# Autodesk Inventor assembly: FA[23]
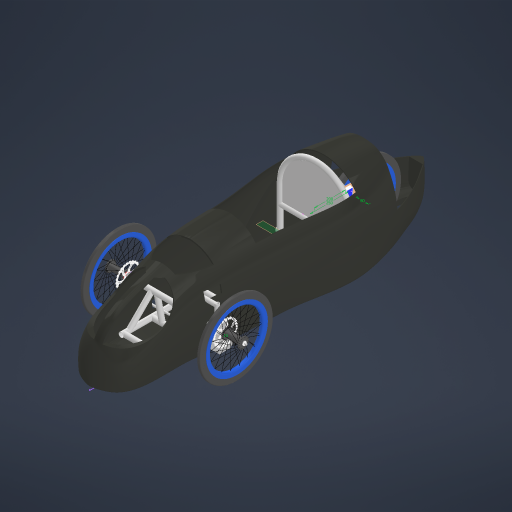
[picture p0: Inventor's stored thumbnail of the model, 512x512]
Saved by Autodesk Inventor 2024 (Build 280153000, 153)
## iProperties
Created: 2023-01-27
Part Number: FA[23]
Document SubType Name: Assembly
Designer: juanj
Author: juanj
## Documents named in this file (22)
- C:\Users\juanj\Documents\Documentos\Unisabana\Shell\A23[F]\FA[23].iam
- C:\Users\juanj\Documents\Documentos\Unisabana\Shell\A23[F]\PFA23[F]\FB23[F].ipt
- C:\Users\juanj\Documents\Documentos\Unisabana\Shell\A23[F]\PFA23[F]\TW23[F].ipt
- C:\Users\juanj\Documents\Documentos\Unisabana\Shell\A23[F]\PFA23[F]\W23[F].ipt
- C:\Users\juanj\Documents\Documentos\Unisabana\Shell\A23[F]\PFA23[F]\BU23[F].ipt
- C:\Users\juanj\Documents\Documentos\Unisabana\Shell\A23[F]\PFA23[F]\C23[F].ipt
- C:\Users\juanj\Documents\Documentos\Unisabana\Shell\A23[F]\PFA23[F]\R23[F].ipt
- C:\Users\juanj\Documents\Documentos\Unisabana\Shell\A23[F]\PFA23[F]\S23[F].ipt
- C:\Users\juanj\Documents\Documentos\Unisabana\Shell\A23[F]\PFA23[F]\N23[1][F].ipt
- C:\Users\juanj\Documents\Documentos\Unisabana\Shell\A23[F]\PFA23[F]\N23[F][2].ipt
- C:\Users\juanj\Documents\Documentos\Unisabana\Shell\A23[F]\PFA23[F]\D23[F].iam
- C:\Users\juanj\Documents\Documentos\Unisabana\Shell\A23[F]\PFA23[F]\M23[F].ipt
- C:\Users\juanj\Documents\Documentos\Unisabana\Shell\A23[F]\PFA23[F]\ET23[F].iam
- C:\Users\juanj\Documents\Documentos\Unisabana\Shell\A23[F]\PFA23[F]\BW23[F].ipt
- C:\Users\juanj\Documents\Documentos\Unisabana\Shell\C23 DESING\A23[F]\PFA23[F]\B23[F]_MIR2.ipt
- C:\Users\juanj\Documents\Documentos\Unisabana\Shell\C23 DESING\A23[F]\PFA23[F]\B23[F1].ipt
- C:\Users\juanj\Documents\Documentos\Unisabana\Shell\C23 DESING\A23[F]\PFA23[F]\HB[F].ipt
- C:\Users\juanj\Documents\Documentos\Unisabana\Shell\C23 DESING\A23[F]\PFA23[F]\C23[i3][L][2].ipt
- C:\Users\juanj\Documents\Documentos\Unisabana\Shell\C23 DESING\A23[F]\PFA23[F]\C23[i3][R][1].ipt
- C:\Users\juanj\Documents\Documentos\Unisabana\Shell\C23 DESING\A23[F]\PFA23[F]\DC23[L][F][1].ipt
- C:\Users\juanj\Documents\Documentos\Unisabana\Shell\C23 DESING\A23[F]\PFA23[F]\DC23[R][F][1].ipt
- C:\Users\juanj\Documents\Documentos\Unisabana\Shell\C23 DESING\A23[F]\PFA23[F]\SW23[F].ipt
## Components (30 placed, 21 different names)
1. C23[F]:1 — Insertar:3
2. FB23[F]:1 — Insertar:3, Insertar:4, Insertar:5, Insertar:6, Insertar:7, Insertar:8, Insertar:37, Nivelación:3, Nivelación:4, Insertar:38, Ángulo:8, Nivelación:5
3. TW23[F]:1 — Insertar:4
4. W23[F]:1 — Insertar:14
5. BU23[F]:1 — Insertar:14, Insertar:21, Insert:47
6. BU23[F]:2 — Insertar:15, Insertar:20, Insert:54
7. R23[F]:1 — Insertar:5, Insert:53
8. R23[F]:2 — Insertar:6
9. R23[F]:3 — Insertar:7
10. R23[F]:4 — Insertar:8, Insert:61
11. W23[F]:2 — Insertar:15
12. S23[F]:1 — Insert:43
13. S23[F]:2 — Insert:49
14. BW23[F]:1 — Insertar:38, Ángulo:8
15. ET23[F]:1 [sub-assembly] — Coincidencia:2, Coincidencia:3, Nivelación:6
16. M23[F]:1 — Insertar:37
17. D23[F]:1 [sub-assembly] — Insert:59, Mate:5
18. N23[F][2]:2 — Insertar:20
19. N23[1][F]:2 — Insert:51
20. N23[F][2]:1 — Insertar:21
21. N23[1][F]:1 — Insert:44
22. HB[F]:1 — Insert:58, Angle:18
23. C23[i3][L][2]:1 — Angle:11, Insert:41, Insert:43, Insert:47, Insert:53, Insert:60, Angle:20
24. C23[i3][R][1]:1 — Insert:49, Angle:14, Insert:50, Insert:54, Angle:17, Insert:61
25. DC23[L][F][1]:1 — Angle:11, Insert:41, Insert:44, Insert:55, Angle:16, Insert:59
26. DC23[R][F][1]:1 — Angle:14, Insert:50, Insert:51, Insert:56, Mate:5
27. B23[F]_MIR2:1 — Insert:56, Angle:17, Insert:58, Angle:18
28. B23[F1]:2 — Insert:55, Angle:16, Insert:57, Angle:19
29. HB[F]:3 — Insert:57, Angle:19
30. SW23[F]:1 — Insert:60, Angle:20
## Relationships (43: Insert 28, Angle 8, Flush 4, Mate 3)
- Insertar:3: C23[F]:1 ↔ FB23[F]:1
- Insertar:4: FB23[F]:1 ↔ TW23[F]:1
- Insertar:5: FB23[F]:1 ↔ R23[F]:1
- Insertar:6: FB23[F]:1 ↔ R23[F]:2
- Insertar:7: FB23[F]:1 ↔ R23[F]:3
- Insertar:8: FB23[F]:1 ↔ R23[F]:4
- Insertar:14: W23[F]:1 ↔ BU23[F]:1
- Insertar:15: BU23[F]:2 ↔ W23[F]:2
- Insertar:20: BU23[F]:2 ↔ N23[F][2]:2
- Insertar:21: BU23[F]:1 ↔ N23[F][2]:1
- Insertar:37: FB23[F]:1 ↔ M23[F]:1
- Nivelación:3 [Flush] (30 mm): FB23[F]:1
- Nivelación:4 [Flush] (29 mm): FB23[F]:1
- Coincidencia:2 [Mate]: ET23[F]:1
- Coincidencia:3 [Mate]: ET23[F]:1
- Insertar:38 (106.5 mm): FB23[F]:1 ↔ BW23[F]:1
- Ángulo:8 [Angle] (180 deg): FB23[F]:1 ↔ BW23[F]:1
- Nivelación:5 [Flush] (-50 mm): FB23[F]:1
- Nivelación:6 [Flush]: ET23[F]:1
- Angle:11 (0 deg): C23[i3][L][2]:1 ↔ DC23[L][F][1]:1
- Insert:41: C23[i3][L][2]:1 ↔ DC23[L][F][1]:1
- Insert:43: S23[F]:1 ↔ C23[i3][L][2]:1
- Insert:44: N23[1][F]:1 ↔ DC23[L][F][1]:1
- Insert:47: BU23[F]:1 ↔ C23[i3][L][2]:1
- Insert:49: S23[F]:2 ↔ C23[i3][R][1]:1
- Angle:14 (0 deg): C23[i3][R][1]:1 ↔ DC23[R][F][1]:1
- Insert:50: C23[i3][R][1]:1 ↔ DC23[R][F][1]:1
- Insert:51: N23[1][F]:2 ↔ DC23[R][F][1]:1
- Insert:53: R23[F]:1 ↔ C23[i3][L][2]:1
- Insert:54: BU23[F]:2 ↔ C23[i3][R][1]:1
- Insert:55: DC23[L][F][1]:1 ↔ B23[F1]:2
- Angle:16 (0 deg): DC23[L][F][1]:1 ↔ B23[F1]:2
- Insert:56: DC23[R][F][1]:1 ↔ B23[F]_MIR2:1
- Angle:17 (0 deg): C23[i3][R][1]:1 ↔ B23[F]_MIR2:1
- Insert:57: B23[F1]:2 ↔ HB[F]:3
- Insert:58: HB[F]:1 ↔ B23[F]_MIR2:1
- Angle:18 (0 deg): HB[F]:1 ↔ B23[F]_MIR2:1
- Angle:19 (0 deg): B23[F1]:2 ↔ HB[F]:3
- Insert:59: D23[F]:1 ↔ DC23[L][F][1]:1
- Insert:60: C23[i3][L][2]:1 ↔ SW23[F]:1
- Angle:20 (0 deg): C23[i3][L][2]:1 ↔ SW23[F]:1
- Insert:61: R23[F]:4 ↔ C23[i3][R][1]:1
- Mate:5: D23[F]:1 ↔ DC23[R][F][1]:1
